# Autodesk Inventor assembly: 203.007.01_ZB_Linearmotor
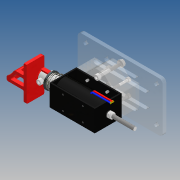
[picture p0: Inventor's stored thumbnail of the model, 180x180]
Saved by Autodesk Inventor 2021 (Build 250183000, 183)
## iProperties
Created: 2021-11-04
Part Number: 203.007.01_ZB_Linearmotor
Document SubType Name: Assembly
Designer: Sebastian Seewald
Author: Sebastian Seewald
## Documents named in this file (16)
- E:\Dokumente\MCI-Mechatronik\Master\Semester_3\Projekt_2_Neu\104_Extrudereinheit\204.005.01_ZB_Hubmagnetstopper.iam
- E:\Dokumente\MCI-Mechatronik\Master\Semester_3\Projekt_2_Neu\104_Extrudereinheit\504.008.01_Hubmagnet_Gehaeuse.ipt
- E:\Dokumente\MCI-Mechatronik\Master\Semester_3\Projekt_2_Neu\104_Extrudereinheit\504.007.01_Anker_Linearmotor.ipt
- E:\Dokumente\MCI-Mechatronik\Master\Semester_3\Projekt_2_Neu\104_Extrudereinheit\104.007.01_Stopper.ipt
- E:\Dokumente\MCI-Mechatronik\Master\Semester_3\Projekt_2_Neu\104_Extrudereinheit\504.009.01_Splint_Feder.ipt
- E:\Dokumente\MCI-Mechatronik\Master\Semester_3\Projekt_2_Neu\104_Extrudereinheit\504.010.01_Feder_Hubmagnet.ipt
- E:\Dokumente\MCI-Mechatronik\Master\Semester_3\Projekt_2_Neu\104_Extrudereinheit\104.008.01_Grundplatte_Stopper.ipt
- E:\Dokumente\MCI-Mechatronik\Master\Semester_3\Projekt_2_Neu\104_Extrudereinheit\104.009.01_Levilierebene_Stopper.ipt
- E:\Dokumente\MCI-Mechatronik\Master\Semester_3\Projekt_2_Neu\104_Extrudereinheit\Schrauben\DIN 934 - M4 x 0.7 Mutter.ipt
- E:\Dokumente\MCI-Mechatronik\Master\Semester_3\Projekt_2_Neu\104_Extrudereinheit\Schrauben\DIN 6902 - M4 Unterlegscheibe.ipt
- E:\Dokumente\MCI-Mechatronik\Master\Semester_3\Projekt_2_Neu\104_Extrudereinheit\Schrauben\DIN 912 - M3 x 30.ipt
- E:\Dokumente\MCI-Mechatronik\Master\Semester_3\Projekt_2_Neu\104_Extrudereinheit\Schrauben\DIN 912 - M4 x 35.ipt
- E:\Dokumente\MCI-Mechatronik\Master\Semester_3\Projekt_2_Neu\104_Extrudereinheit\Schrauben\ISO 10511 - M5 x 05 Mutter.ipt
- E:\Dokumente\MCI-Mechatronik\Master\Semester_3\Projekt_2_Neu\104_Extrudereinheit\Schrauben\DIN 912 - M4 x 20.ipt
- E:\Dokumente\MCI-Mechatronik\Master\Semester_3\Projekt_2_Neu\104_Extrudereinheit\104.012.01_Gummiring_Hubmagnet.ipt
- E:\Dokumente\MCI-Mechatronik\Master\Semester_3\Projekt_2_Neu\104_Extrudereinheit\104.013.01_Daempfer_Stopper.ipt
## Components (27 placed, 15 different names)
1. 504.008.01_Hubmagnet_Gehaeuse:1 — Passend:1, Winkel:1, Federweg, Passend:10, Passend:60, Fluchtend:6, Fluchtend:7, Fluchtend:8, Fluchtend:9, Fluchtend:10, Fluchtend:11, Fluchtend:12, Fluchtend:13, Fluchtend:14, Fluchtend:15, Passend:77, Passend:78, Passend:79, Passend:80, Winkel:3, Fluchtend:16
2. 504.007.01_Anker_Linearmotor:1 — Passend:1, Passend:2, Winkel:1, Passend:3, Winkel:2, Passend:5, Passend:6, Passend:8, Passend:73, Passend:74, Tangential:1, Tangential:2, Passend:88, Fluchtend:17
3. 104.007.01_Stopper:1 — Passend:2, Passend:3, Winkel:2, Passend:89, Passend:90, Passend:91, Passend:92, Passend:93, Passend:94
4. DIN 912 - M4 x 20:1 — Passend:74, Tangential:1, Passend:75
5. DIN 934 - M4 x 0.7 Mutter:3 — Passend:75, Tangential:2
6. 504.009.01_Splint_Feder:1 — Passend:5, Passend:6, Federweg, Passend:9
7. 504.010.01_Feder_Hubmagnet:1 — Passend:8, Passend:9, Passend:10
8. 104.008.01_Grundplatte_Stopper:1 — Passend:23, Passend:50, Passend:51, Winkel:3, Passend:83, Fluchtend:16
9. 104.009.01_Levilierebene_Stopper:1 — Passend:20, Passend:23, Passend:67, Passend:68, Passend:69, Passend:70, Fluchtend:14, Fluchtend:15
10. 104.009.01_Levilierebene_Stopper:3 — Passend:17, Passend:20, Fluchtend:6, Fluchtend:7
11. 104.009.01_Levilierebene_Stopper:2 — Passend:17, Passend:54, Fluchtend:8, Fluchtend:9
12. 104.009.01_Levilierebene_Stopper:4 — Passend:54, Passend:59, Fluchtend:10, Fluchtend:11
13. 104.009.01_Levilierebene_Stopper:5 — Passend:59, Passend:60, Passend:71, Passend:72, Fluchtend:12, Fluchtend:13, Passend:81, Passend:82
14. DIN 934 - M4 x 0.7 Mutter:1 — Passend:52, Passend:85
15. DIN 934 - M4 x 0.7 Mutter:2 — Passend:53, Passend:87
16. DIN 6902 - M4 Unterlegscheibe:1 — Passend:51, Passend:52, Passend:84
17. DIN 6902 - M4 Unterlegscheibe:2 — Passend:50, Passend:53, Passend:86
18. DIN 912 - M3 x 30:1 — Passend:70, Passend:80
19. DIN 912 - M3 x 30:2 — Passend:68, Passend:79
20. DIN 912 - M3 x 30:3 — Passend:69, Passend:77
21. DIN 912 - M3 x 30:4 — Passend:67, Passend:78
22. DIN 912 - M4 x 35:1 — Passend:71, Passend:81, Passend:86, Passend:87
23. DIN 912 - M4 x 35:2 — Passend:72, Passend:82, Passend:83, Passend:84, Passend:85
24. ISO 10511 - M5 x 05 Mutter:1 — Passend:73, Fluchtend:17, Tangential:3
25. 104.012.01_Gummiring_Hubmagnet:1 — Passend:88, Tangential:3
26. 104.013.01_Daempfer_Stopper:1 — Passend:89, Passend:90, Passend:91
27. 104.013.01_Daempfer_Stopper:2 — Passend:92, Passend:93, Passend:94
## Relationships (64: Mate 46, Flush 12, Angle 3, Tangent 3)
- Passend:1 [Mate]: 504.008.01_Hubmagnet_Gehaeuse:1 ↔ 504.007.01_Anker_Linearmotor:1
- Passend:2 [Mate]: 504.007.01_Anker_Linearmotor:1 ↔ 104.007.01_Stopper:1
- Winkel:1 [Angle] (270 deg): 504.008.01_Hubmagnet_Gehaeuse:1 ↔ 504.007.01_Anker_Linearmotor:1
- Passend:3 [Mate]: 504.007.01_Anker_Linearmotor:1 ↔ 104.007.01_Stopper:1
- Winkel:2 [Angle] (0 deg): 504.007.01_Anker_Linearmotor:1 ↔ 104.007.01_Stopper:1
- Passend:5 [Mate]: 504.007.01_Anker_Linearmotor:1 ↔ 504.009.01_Splint_Feder:1
- Passend:6 [Mate]: 504.007.01_Anker_Linearmotor:1 ↔ 504.009.01_Splint_Feder:1
- Federweg [Mate] (15 mm): 504.008.01_Hubmagnet_Gehaeuse:1 ↔ 504.009.01_Splint_Feder:1
- Passend:8 [Mate]: 504.007.01_Anker_Linearmotor:1 ↔ 504.010.01_Feder_Hubmagnet:1
- Passend:9 [Mate]: 504.009.01_Splint_Feder:1 ↔ 504.010.01_Feder_Hubmagnet:1
- Passend:10 [Mate]: 504.008.01_Hubmagnet_Gehaeuse:1 ↔ 504.010.01_Feder_Hubmagnet:1
- Passend:17 [Mate]: 104.009.01_Levilierebene_Stopper:3 ↔ 104.009.01_Levilierebene_Stopper:2
- Passend:20 [Mate]: 104.009.01_Levilierebene_Stopper:1 ↔ 104.009.01_Levilierebene_Stopper:3
- Passend:23 [Mate]: 104.008.01_Grundplatte_Stopper:1 ↔ 104.009.01_Levilierebene_Stopper:1
- Passend:50 [Mate]: 104.008.01_Grundplatte_Stopper:1 ↔ DIN 6902 - M4 Unterlegscheibe:2
- Passend:51 [Mate]: 104.008.01_Grundplatte_Stopper:1 ↔ DIN 6902 - M4 Unterlegscheibe:1
- Passend:52 [Mate]: DIN 934 - M4 x 0.7 Mutter:1 ↔ DIN 6902 - M4 Unterlegscheibe:1
- Passend:53 [Mate]: DIN 934 - M4 x 0.7 Mutter:2 ↔ DIN 6902 - M4 Unterlegscheibe:2
- Passend:54 [Mate]: 104.009.01_Levilierebene_Stopper:2 ↔ 104.009.01_Levilierebene_Stopper:4
- Passend:59 [Mate]: 104.009.01_Levilierebene_Stopper:4 ↔ 104.009.01_Levilierebene_Stopper:5
- Passend:60 [Mate]: 504.008.01_Hubmagnet_Gehaeuse:1 ↔ 104.009.01_Levilierebene_Stopper:5
- Passend:67 [Mate]: 104.009.01_Levilierebene_Stopper:1 ↔ DIN 912 - M3 x 30:4
- Passend:68 [Mate]: 104.009.01_Levilierebene_Stopper:1 ↔ DIN 912 - M3 x 30:2
- Passend:69 [Mate]: 104.009.01_Levilierebene_Stopper:1 ↔ DIN 912 - M3 x 30:3
- Passend:70 [Mate]: 104.009.01_Levilierebene_Stopper:1 ↔ DIN 912 - M3 x 30:1
- Passend:71 [Mate]: 104.009.01_Levilierebene_Stopper:5 ↔ DIN 912 - M4 x 35:1
- Passend:72 [Mate]: 104.009.01_Levilierebene_Stopper:5 ↔ DIN 912 - M4 x 35:2
- Passend:73 [Mate]: 504.007.01_Anker_Linearmotor:1 ↔ ISO 10511 - M5 x 05 Mutter:1
- Passend:74 [Mate]: 504.007.01_Anker_Linearmotor:1 ↔ DIN 912 - M4 x 20:1
- Tangential:1: 504.007.01_Anker_Linearmotor:1 ↔ DIN 912 - M4 x 20:1
- Passend:75 [Mate]: DIN 912 - M4 x 20:1 ↔ DIN 934 - M4 x 0.7 Mutter:3
- Tangential:2: 504.007.01_Anker_Linearmotor:1 ↔ DIN 934 - M4 x 0.7 Mutter:3
- Fluchtend:6 [Flush]: 504.008.01_Hubmagnet_Gehaeuse:1 ↔ 104.009.01_Levilierebene_Stopper:3
- Fluchtend:7 [Flush]: 504.008.01_Hubmagnet_Gehaeuse:1 ↔ 104.009.01_Levilierebene_Stopper:3
- Fluchtend:8 [Flush]: 504.008.01_Hubmagnet_Gehaeuse:1 ↔ 104.009.01_Levilierebene_Stopper:2
- Fluchtend:9 [Flush]: 504.008.01_Hubmagnet_Gehaeuse:1 ↔ 104.009.01_Levilierebene_Stopper:2
- Fluchtend:10 [Flush]: 504.008.01_Hubmagnet_Gehaeuse:1 ↔ 104.009.01_Levilierebene_Stopper:4
- Fluchtend:11 [Flush]: 504.008.01_Hubmagnet_Gehaeuse:1 ↔ 104.009.01_Levilierebene_Stopper:4
- Fluchtend:12 [Flush]: 504.008.01_Hubmagnet_Gehaeuse:1 ↔ 104.009.01_Levilierebene_Stopper:5
- Fluchtend:13 [Flush]: 504.008.01_Hubmagnet_Gehaeuse:1 ↔ 104.009.01_Levilierebene_Stopper:5
- Fluchtend:14 [Flush]: 504.008.01_Hubmagnet_Gehaeuse:1 ↔ 104.009.01_Levilierebene_Stopper:1
- Fluchtend:15 [Flush]: 504.008.01_Hubmagnet_Gehaeuse:1 ↔ 104.009.01_Levilierebene_Stopper:1
- Passend:77 [Mate]: 504.008.01_Hubmagnet_Gehaeuse:1 ↔ DIN 912 - M3 x 30:3
- Passend:78 [Mate]: 504.008.01_Hubmagnet_Gehaeuse:1 ↔ DIN 912 - M3 x 30:4
- Passend:79 [Mate]: 504.008.01_Hubmagnet_Gehaeuse:1 ↔ DIN 912 - M3 x 30:2
- Passend:80 [Mate]: 504.008.01_Hubmagnet_Gehaeuse:1 ↔ DIN 912 - M3 x 30:1
- Passend:81 [Mate]: 104.009.01_Levilierebene_Stopper:5 ↔ DIN 912 - M4 x 35:1
- Passend:82 [Mate]: 104.009.01_Levilierebene_Stopper:5 ↔ DIN 912 - M4 x 35:2
- Winkel:3 [Angle] (0 deg): 504.008.01_Hubmagnet_Gehaeuse:1 ↔ 104.008.01_Grundplatte_Stopper:1
- Passend:83 [Mate] (2.5 mm): 104.008.01_Grundplatte_Stopper:1 ↔ DIN 912 - M4 x 35:2
- Passend:84 [Mate]: DIN 6902 - M4 Unterlegscheibe:1 ↔ DIN 912 - M4 x 35:2
- Passend:85 [Mate]: DIN 934 - M4 x 0.7 Mutter:1 ↔ DIN 912 - M4 x 35:2
- Passend:86 [Mate]: DIN 6902 - M4 Unterlegscheibe:2 ↔ DIN 912 - M4 x 35:1
- Passend:87 [Mate]: DIN 934 - M4 x 0.7 Mutter:2 ↔ DIN 912 - M4 x 35:1
- Fluchtend:16 [Flush] (33 mm): 504.008.01_Hubmagnet_Gehaeuse:1 ↔ 104.008.01_Grundplatte_Stopper:1
- Passend:88 [Mate]: 504.007.01_Anker_Linearmotor:1 ↔ 104.012.01_Gummiring_Hubmagnet:1
- Fluchtend:17 [Flush] (-31 mm): 504.007.01_Anker_Linearmotor:1 ↔ ISO 10511 - M5 x 05 Mutter:1
- Tangential:3: ISO 10511 - M5 x 05 Mutter:1 ↔ 104.012.01_Gummiring_Hubmagnet:1
- Passend:89 [Mate]: 104.007.01_Stopper:1 ↔ 104.013.01_Daempfer_Stopper:1
- Passend:90 [Mate]: 104.007.01_Stopper:1 ↔ 104.013.01_Daempfer_Stopper:1
- Passend:91 [Mate]: 104.007.01_Stopper:1 ↔ 104.013.01_Daempfer_Stopper:1
- Passend:92 [Mate]: 104.007.01_Stopper:1 ↔ 104.013.01_Daempfer_Stopper:2
- Passend:93 [Mate]: 104.007.01_Stopper:1 ↔ 104.013.01_Daempfer_Stopper:2
- Passend:94 [Mate]: 104.007.01_Stopper:1 ↔ 104.013.01_Daempfer_Stopper:2
